# Autodesk Inventor assembly: ASY ДМФ 0100 Барабан v2.1
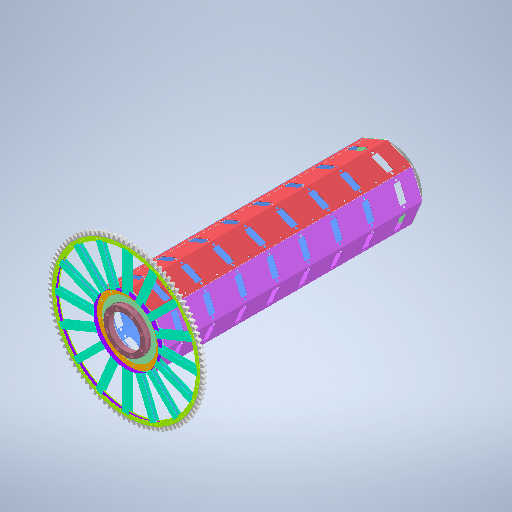
[picture p0: Inventor's stored thumbnail of the model, 512x512]
Saved by Autodesk Inventor 2025 (Build 290162010, 162A)
## iProperties
Created: 2024-04-28
Part Number: ASY ДМФ 0100 Барабан v2.1
Document SubType Name: Assembly
Designer: pokla
Author: pokla
## Documents named in this file (20)
- C:\Users\pokla\Documents\Inventor\ДФО\ДМФ\DMF-Disk-Micro-Filter\Барабан v2.1\ASY ДМФ 0100 Барабан v2.1.iam
- C:\Users\pokla\Documents\Inventor\ДФО\ДМФ\DMF-Disk-Micro-Filter\Барабан v2.1\DMF 01 21 Барабан торец НОС v2.1.ipt
- C:\Users\pokla\Documents\Inventor\ДФО\ДМФ\DMF-Disk-Micro-Filter\Барабан v2.1\DMF 01 13 Барабан Лист лев брт v2.1.ipt
- C:\Users\pokla\Documents\Inventor\ДФО\ДМФ\DMF-Disk-Micro-Filter\Барабан v2.1\DMF 01 14 Барабан Лист прав брт v2.1.ipt
- C:\Users\pokla\Documents\Inventor\ДФО\ДМФ\DMF-Disk-Micro-Filter\Барабан v2.1\DMF 01 31 Барабан Опорное кольцо НОС v2.1.ipt
- C:\Users\pokla\Documents\Inventor\ДФО\ДМФ\DMF-Disk-Micro-Filter\Барабан v2.1\DMF 01 17 опора крышки v2.1.ipt
- C:\Users\pokla\Documents\Inventor\ДФО\ДМФ\DMF-Disk-Micro-Filter\Барабан v2.1\DMF 000 размеры v2.1.ipt
- C:\Users\pokla\Documents\Inventor\ДФО\ДМФ\DMF-Disk-Micro-Filter\Барабан v2.1\DMF 01 12 Барабан усилитель v2.1.ipt
- C:\Users\pokla\Documents\Inventor\ДФО\ДМФ\DMF-Disk-Micro-Filter\Барабан v2.1\ASY DMF 010 cap v2.1.iam
- C:\Users\pokla\Documents\Inventor\ДФО\ДМФ\DMF-Disk-Micro-Filter\Барабан v2.1\DMF 01 32 Барабан Опорное кольцо КОРМА v2.1.ipt
- C:\Users\pokla\Documents\Inventor\ДФО\ДМФ\DMF-Disk-Micro-Filter\Барабан v2.1\DMF 01 22 Барабан торец КОРМА v2.1.ipt
- C:\Users\pokla\Documents\Inventor\ДФО\ДМФ\DMF-Disk-Micro-Filter\Барабан v2.1\ASY DMF filter package v2.1.iam
- C:\Users\pokla\Documents\Inventor\ДФО\ДМФ\DMF-Disk-Micro-Filter\Барабан v2.1\DMF 01 21 cylinder butt end nose.ipt
- C:\Users\pokla\Documents\Inventor\ДФО\ДМФ\DMF-Disk-Micro-Filter\Барабан v2.1\DMF 2.1 01 42 Gear way 2.ipt
- C:\Users\pokla\Documents\Inventor\ДФО\ДМФ\DMF-Disk-Micro-Filter\Барабан v2.1\DMF 2.1 01 43 Gear rim 3.ipt
- C:\Users\pokla\Documents\Inventor\ДФО\ДМФ\DMF-Disk-Micro-Filter\Барабан v2.1\DMF 2.1 01 44 Gear rim 4.ipt
- C:\Users\pokla\Documents\Inventor\ДФО\ДМФ\DMF-Disk-Micro-Filter\Барабан v2.1\DMF 2.1 01 45 Gear ring 5.ipt
- C:\Users\pokla\Documents\Inventor\ДФО\ДМФ\DMF-Disk-Micro-Filter\Барабан v2.1\DMF 2.1 01 46 Gear axis wheel 6.ipt
- C:\Users\pokla\Documents\Inventor\ДФО\ДМФ\DMF-Disk-Micro-Filter\Барабан v2.1\DMF 01 13 Барабан усилитель v2.1.ipt
- C:\Users\pokla\Documents\Inventor\ДФО\ДМФ\DMF-Disk-Micro-Filter\шестерни 06.09.2025\DMF sector big gear 2.1.ipt
## Components (104 placed, 19 different names)
1. DMF 000 размеры v2.1.ipt:1 — Rigid:30
2. DMF 01 21 Барабан торец НОС v2.1.ipt:1 — Mate:15, Flush:8, Flush:9, Flush:10, Flush:11, Mate:16, Mate:17, Mate:19, Mate:21, Flush:15, Flush:16, Flush:17, Mate:23, Rigid:27, Rigid:29, Rigid:30, Rigid:34
3. DMF 01 31 Барабан Опорное кольцо НОС v2.1.ipt:1 — Rigid:29
4. DMF 01 32 Барабан Опорное кольцо КОРМА v2.1.ipt:1 — Rigid:20
5. DMF 01 22 Барабан торец КОРМА v2.1.ipt:1 — Flush:12, Flush:13, Mate:18, Rigid:20
6. DMF 01 13 Барабан Лист лев брт v2.1.ipt:1 — Flush:10, Flush:11, Mate:16, Flush:13, Mate:18, Mate:20, Mate:29
7. DMF 01 14 Барабан Лист прав брт v2.1.ipt:1 — Flush:8, Flush:9, Mate:17, Flush:12, Mate:22, Mate:28
8. DMF 01 17 опора крышки v2.1.ipt:1 — Mate:21, Flush:15, Mate:22
9. DMF 01 17 опора крышки v2.1.ipt:2 — Mate:19, Mate:20, Mate:27
10. ASY DMF 010 cap v2.1.iam:1 [sub-assembly] — Flush:16, Flush:17, Mate:23, Mate:27
11. DMF 01 21 cylinder butt end nose.ipt:1 — Mate:28, Mate:29
12. DMF 2.1 01 45 Gear ring 5.ipt:1 — Rigid:21, Rigid:22, Rigid:23, Rigid:27, Rigid:31
13. DMF 2.1 01 46 Gear axis wheel 6.ipt:1 — Rigid:31
14. ASY DMF filter package v2.1.iam:1 [sub-assembly] — Mate:24, Mate:25
15. ASY DMF filter package v2.1.iam:2 [sub-assembly]
16. ASY DMF filter package v2.1.iam:3 [sub-assembly]
17. ASY DMF filter package v2.1.iam:4 [sub-assembly]
18. ASY DMF filter package v2.1.iam:5 [sub-assembly]
19. ASY DMF filter package v2.1.iam:6 [sub-assembly]
20. ASY DMF filter package v2.1.iam:7 [sub-assembly]
21. ASY DMF filter package v2.1.iam:8 [sub-assembly]
22. DMF 2.1 01 43 Gear rim 3.ipt:1 — Rigid:24
23. DMF 2.1 01 43 Gear rim 3.ipt:2 — Rigid:23, Rigid:24
24. DMF 2.1 01 43 Gear rim 3.ipt:3
25. DMF 2.1 01 43 Gear rim 3.ipt:4
26. DMF 2.1 01 43 Gear rim 3.ipt:5
27. DMF 2.1 01 43 Gear rim 3.ipt:6
28. DMF 2.1 01 43 Gear rim 3.ipt:7
29. DMF 2.1 01 43 Gear rim 3.ipt:8
30. DMF 2.1 01 44 Gear rim 4.ipt:1 — Rigid:22
31. DMF 2.1 01 44 Gear rim 4.ipt:2
32. DMF 2.1 01 44 Gear rim 4.ipt:3
33. DMF 01 12 Барабан усилитель v2.1.ipt:1 — Mate:30, Tangent:1, Mate:31, Rigid:21, Flush:18, Mate:32, Mate:33
34. DMF 2.1 01 42 Gear way 2.ipt:1 — Mate:30, Tangent:1, Mate:31
35. DMF 01 13 Барабан усилитель v2.1.ipt:1 — Flush:18, Mate:32, Mate:33
36. DMF 01 12 Барабан усилитель v2.1.ipt:2
37. DMF 2.1 01 42 Gear way 2.ipt:2
38. DMF 01 13 Барабан усилитель v2.1.ipt:2
39. DMF 01 12 Барабан усилитель v2.1.ipt:3
40. DMF 2.1 01 42 Gear way 2.ipt:3
41. DMF 01 13 Барабан усилитель v2.1.ipt:3
42. DMF 01 12 Барабан усилитель v2.1.ipt:4
43. DMF 2.1 01 42 Gear way 2.ipt:4
44. DMF 01 13 Барабан усилитель v2.1.ipt:4
45. DMF 01 12 Барабан усилитель v2.1.ipt:5
46. DMF 2.1 01 42 Gear way 2.ipt:5
47. DMF 01 13 Барабан усилитель v2.1.ipt:5
48. DMF 01 12 Барабан усилитель v2.1.ipt:6
49. DMF 2.1 01 42 Gear way 2.ipt:6
50. DMF 01 13 Барабан усилитель v2.1.ipt:6
51. DMF 01 12 Барабан усилитель v2.1.ipt:7
52. DMF 2.1 01 42 Gear way 2.ipt:7
53. DMF 01 13 Барабан усилитель v2.1.ipt:7
54. DMF 01 12 Барабан усилитель v2.1.ipt:8
55. DMF 2.1 01 42 Gear way 2.ipt:8
56. DMF 01 13 Барабан усилитель v2.1.ipt:8
57. DMF 01 12 Барабан усилитель v2.1.ipt:9
58. DMF 2.1 01 42 Gear way 2.ipt:9
59. DMF 01 13 Барабан усилитель v2.1.ipt:9
60. DMF 01 12 Барабан усилитель v2.1.ipt:10
61. DMF 2.1 01 42 Gear way 2.ipt:10
62. DMF 01 13 Барабан усилитель v2.1.ipt:10
63. DMF 01 12 Барабан усилитель v2.1.ipt:11
64. DMF 2.1 01 42 Gear way 2.ipt:11
65. DMF 01 13 Барабан усилитель v2.1.ipt:11
66. DMF 01 12 Барабан усилитель v2.1.ipt:12
67. DMF 2.1 01 42 Gear way 2.ipt:12
68. DMF 01 13 Барабан усилитель v2.1.ipt:12
69. DMF 01 12 Барабан усилитель v2.1.ipt:13
70. DMF 2.1 01 42 Gear way 2.ipt:13
71. DMF 01 13 Барабан усилитель v2.1.ipt:13
72. DMF 01 12 Барабан усилитель v2.1.ipt:14
73. DMF 2.1 01 42 Gear way 2.ipt:14
74. DMF 01 13 Барабан усилитель v2.1.ipt:14
75. DMF 01 12 Барабан усилитель v2.1.ipt:15
76. DMF 2.1 01 42 Gear way 2.ipt:15
77. DMF 01 13 Барабан усилитель v2.1.ipt:15
78. DMF 01 12 Барабан усилитель v2.1.ipt:16
79. DMF 2.1 01 42 Gear way 2.ipt:16
80. DMF 01 13 Барабан усилитель v2.1.ipt:16
81. DMF sector big gear 2.1.ipt:1 — Rigid:34
82. DMF sector big gear 2.1.ipt:2
83. DMF sector big gear 2.1.ipt:3
84. DMF sector big gear 2.1.ipt:4
85. DMF sector big gear 2.1.ipt:5
86. DMF sector big gear 2.1.ipt:6
87. DMF sector big gear 2.1.ipt:7
88. DMF sector big gear 2.1.ipt:8
89. DMF sector big gear 2.1.ipt:9
90. DMF sector big gear 2.1.ipt:10
91. DMF sector big gear 2.1.ipt:11
92. DMF sector big gear 2.1.ipt:12
93. DMF sector big gear 2.1.ipt:13
94. DMF sector big gear 2.1.ipt:14
95. DMF sector big gear 2.1.ipt:15
96. DMF sector big gear 2.1.ipt:16
97. DMF sector big gear 2.1.ipt:17
98. DMF sector big gear 2.1.ipt:18
99. DMF sector big gear 2.1.ipt:19
100. DMF sector big gear 2.1.ipt:20
101. DMF sector big gear 2.1.ipt:21
102. DMF sector big gear 2.1.ipt:22
103. DMF sector big gear 2.1.ipt:23
104. DMF sector big gear 2.1.ipt:24
## Component patterns: (8 elements, first: ASY DMF filter package v2.1.iam:1), (4 elements, first: DMF 2.1 01 43 Gear rim 3.ipt:1 + DMF 2.1 01 43 Gear rim 3.ipt:2), (3 elements, first: DMF 2.1 01 44 Gear rim 4.ipt:1), (16 elements, first: DMF 01 12 Барабан усилитель v2.1.ipt:1 + DMF 2.1 01 42 Gear way 2.ipt:1 + DMF 01 13 Барабан усилитель v2.1.ipt:1), (24 elements, first: DMF sector big gear 2.1.ipt:1)
## Relationships (39: Mate 18, Flush 10, WeldJoint 10, Tangent 1)
- Mate:15: DMF 01 21 Барабан торец НОС v2.1.ipt:1
- Flush:8: DMF 01 21 Барабан торец НОС v2.1.ipt:1 ↔ DMF 01 14 Барабан Лист прав брт v2.1.ipt:1
- Flush:9: DMF 01 21 Барабан торец НОС v2.1.ipt:1 ↔ DMF 01 14 Барабан Лист прав брт v2.1.ipt:1
- Flush:10: DMF 01 21 Барабан торец НОС v2.1.ipt:1 ↔ DMF 01 13 Барабан Лист лев брт v2.1.ipt:1
- Flush:11: DMF 01 21 Барабан торец НОС v2.1.ipt:1 ↔ DMF 01 13 Барабан Лист лев брт v2.1.ipt:1
- Mate:16: DMF 01 21 Барабан торец НОС v2.1.ipt:1 ↔ DMF 01 13 Барабан Лист лев брт v2.1.ipt:1
- Mate:17: DMF 01 21 Барабан торец НОС v2.1.ipt:1 ↔ DMF 01 14 Барабан Лист прав брт v2.1.ipt:1
- Flush:12: DMF 01 22 Барабан торец КОРМА v2.1.ipt:1 ↔ DMF 01 14 Барабан Лист прав брт v2.1.ipt:1
- Flush:13: DMF 01 22 Барабан торец КОРМА v2.1.ipt:1 ↔ DMF 01 13 Барабан Лист лев брт v2.1.ipt:1
- Mate:18: DMF 01 22 Барабан торец КОРМА v2.1.ipt:1 ↔ DMF 01 13 Барабан Лист лев брт v2.1.ipt:1
- Mate:19: DMF 01 21 Барабан торец НОС v2.1.ipt:1 ↔ DMF 01 17 опора крышки v2.1.ipt:2
- Mate:20: DMF 01 13 Барабан Лист лев брт v2.1.ipt:1 ↔ DMF 01 17 опора крышки v2.1.ipt:2
- Mate:21: DMF 01 21 Барабан торец НОС v2.1.ipt:1 ↔ DMF 01 17 опора крышки v2.1.ipt:1
- Flush:15 (-2 mm): DMF 01 21 Барабан торец НОС v2.1.ipt:1 ↔ DMF 01 17 опора крышки v2.1.ipt:1
- Mate:22: DMF 01 14 Барабан Лист прав брт v2.1.ipt:1 ↔ DMF 01 17 опора крышки v2.1.ipt:1
- Flush:16: DMF 01 21 Барабан торец НОС v2.1.ipt:1 ↔ ASY DMF 010 cap v2.1.iam:1
- Flush:17: DMF 01 21 Барабан торец НОС v2.1.ipt:1 ↔ ASY DMF 010 cap v2.1.iam:1
- Mate:23: DMF 01 21 Барабан торец НОС v2.1.ipt:1 ↔ ASY DMF 010 cap v2.1.iam:1
- Mate:24: ASY DMF filter package v2.1.iam:1
- Mate:25: ASY DMF filter package v2.1.iam:1
- Mate:27: DMF 01 17 опора крышки v2.1.ipt:2 ↔ ASY DMF 010 cap v2.1.iam:1
- Mate:28: DMF 01 14 Барабан Лист прав брт v2.1.ipt:1 ↔ DMF 01 21 cylinder butt end nose.ipt:1
- Mate:29: DMF 01 13 Барабан Лист лев брт v2.1.ipt:1 ↔ DMF 01 21 cylinder butt end nose.ipt:1
- Rigid:20 [WeldJoint]: DMF 01 32 Барабан Опорное кольцо КОРМА v2.1.ipt:1 ↔ DMF 01 22 Барабан торец КОРМА v2.1.ipt:1
- Mate:30: DMF 01 12 Барабан усилитель v2.1.ipt:1 ↔ DMF 2.1 01 42 Gear way 2.ipt:1
- Tangent:1: DMF 01 12 Барабан усилитель v2.1.ipt:1 ↔ DMF 2.1 01 42 Gear way 2.ipt:1
- Mate:31: DMF 01 12 Барабан усилитель v2.1.ipt:1 ↔ DMF 2.1 01 42 Gear way 2.ipt:1
- Rigid:21 [WeldJoint]: DMF 2.1 01 45 Gear ring 5.ipt:1 ↔ DMF 01 12 Барабан усилитель v2.1.ipt:1
- Rigid:22 [WeldJoint]: DMF 2.1 01 45 Gear ring 5.ipt:1 ↔ DMF 2.1 01 44 Gear rim 4.ipt:1
- Rigid:23 [WeldJoint]: DMF 2.1 01 45 Gear ring 5.ipt:1 ↔ DMF 2.1 01 43 Gear rim 3.ipt:2
- Rigid:24 [WeldJoint] (25 mm): DMF 2.1 01 43 Gear rim 3.ipt:1 ↔ DMF 2.1 01 43 Gear rim 3.ipt:2
- Rigid:27 [WeldJoint]: DMF 01 21 Барабан торец НОС v2.1.ipt:1 ↔ DMF 2.1 01 45 Gear ring 5.ipt:1
- Rigid:29 [WeldJoint]: DMF 01 21 Барабан торец НОС v2.1.ipt:1 ↔ DMF 01 31 Барабан Опорное кольцо НОС v2.1.ipt:1
- Rigid:30 [WeldJoint]: DMF 000 размеры v2.1.ipt:1 ↔ DMF 01 21 Барабан торец НОС v2.1.ipt:1
- Rigid:31 [WeldJoint]: DMF 2.1 01 45 Gear ring 5.ipt:1 ↔ DMF 2.1 01 46 Gear axis wheel 6.ipt:1
- Flush:18: DMF 01 12 Барабан усилитель v2.1.ipt:1 ↔ DMF 01 13 Барабан усилитель v2.1.ipt:1
- Mate:32 (2 mm): DMF 01 12 Барабан усилитель v2.1.ipt:1 ↔ DMF 01 13 Барабан усилитель v2.1.ipt:1
- Mate:33 (27 mm): DMF 01 12 Барабан усилитель v2.1.ipt:1 ↔ DMF 01 13 Барабан усилитель v2.1.ipt:1
- Rigid:34 [WeldJoint] (2.5 mm): DMF 01 21 Барабан торец НОС v2.1.ipt:1 ↔ DMF sector big gear 2.1.ipt:1
